# Autodesk Inventor assembly: RA_haz
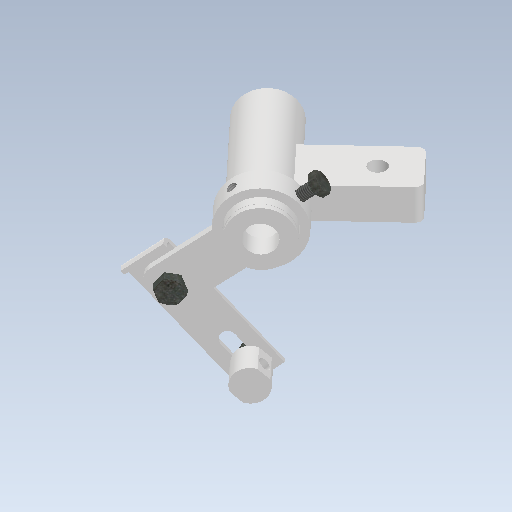
[picture p0: Inventor's stored thumbnail of the model, 512x512]
Saved by Autodesk Inventor 2021.4 (Build 254397000, 397)
## iProperties
Created: 2023-12-02
Part Number: RA_haz
Document SubType Name: Assembly
Designer: vtoth
Author: vtoth
## Documents named in this file (10)
- C:\Users\vtoth\OneDrive - Budapesti Műszaki és Gazdaságtudományi Egyetem\5_felev\CAD\hf2_v2\RA_haz.iam
- C:\Users\vtoth\OneDrive - Budapesti Műszaki és Gazdaságtudományi Egyetem\5_felev\CAD\hf2_v2\ra_haz_1.ipt
- C:\Users\vtoth\OneDrive - Budapesti Műszaki és Gazdaságtudományi Egyetem\5_felev\CAD\hf2_v2\ra_veg.ipt
- C:\Users\vtoth\OneDrive - Budapesti Műszaki és Gazdaságtudományi Egyetem\5_felev\CAD\hf2_v2\ra_kar1.ipt
- C:\Users\vtoth\OneDrive - Budapesti Műszaki és Gazdaságtudományi Egyetem\5_felev\CAD\hf2_v2\ra_kar2.ipt
- C:\Users\vtoth\OneDrive - Budapesti Műszaki és Gazdaságtudományi Egyetem\5_felev\CAD\hf2_v2\ra_csapagy.ipt
- C:\Users\vtoth\OneDrive - Budapesti Műszaki és Gazdaságtudományi Egyetem\5_felev\CAD\hf2_v2\ContentCenter\en-US\ISO 4018\ISO 4018 - M8 x 16.ipt
- C:\Users\vtoth\OneDrive - Budapesti Műszaki és Gazdaságtudományi Egyetem\5_felev\CAD\hf2_v2\ContentCenter\en-US\ISO 4018\ISO 4018 - M10 x 20.ipt
- C:\Users\vtoth\OneDrive - Budapesti Műszaki és Gazdaságtudományi Egyetem\5_felev\CAD\hf2_v2\ContentCenter\en-US\ISO 4032(2)\ISO 4032 - M10 - ISO.ipt
- C:\Users\vtoth\OneDrive - Budapesti Műszaki és Gazdaságtudományi Egyetem\5_felev\CAD\hf2_v2\ContentCenter\en-US\ISO 4036(2)\ISO 4036 - M10(2).ipt
## Components (9 placed, 9 different names)
1. ra_haz_1:1 — Mate:1, Insert:1, Tangent:1
2. ra_veg:1 — Insert:1
3. ra_kar1:1 — Mate:1, Insert:3, Mate:2, Insert:4
4. ra_kar2:1 — Insert:2, Insert:3, Insert:5, Insert:6
5. ra_csapagy:1 — Insert:2
6. ISO 4018 M8 x 16:1 — Mate:2, Tangent:1
7. ISO 4018 M10 x 20:1 — Insert:4
8. ISO 4032 M10:1 — Insert:5
9. ISO 4036 M10:1 — Insert:6
## Relationships (9: Insert 6, Mate 2, Tangent 1)
- Mate:1: ra_haz_1:1 ↔ ra_kar1:1
- Insert:1: ra_haz_1:1 ↔ ra_veg:1
- Insert:2: ra_kar2:1 ↔ ra_csapagy:1
- Insert:3: ra_kar1:1 ↔ ra_kar2:1
- Mate:2: ra_kar1:1 ↔ ISO 4018 M8 x 16:1
- Tangent:1: ra_haz_1:1 ↔ ISO 4018 M8 x 16:1
- Insert:4: ra_kar1:1 ↔ ISO 4018 M10 x 20:1
- Insert:5: ra_kar2:1 ↔ ISO 4032 M10:1
- Insert:6: ra_kar2:1 ↔ ISO 4036 M10:1
